# Autodesk Inventor assembly: tower_half
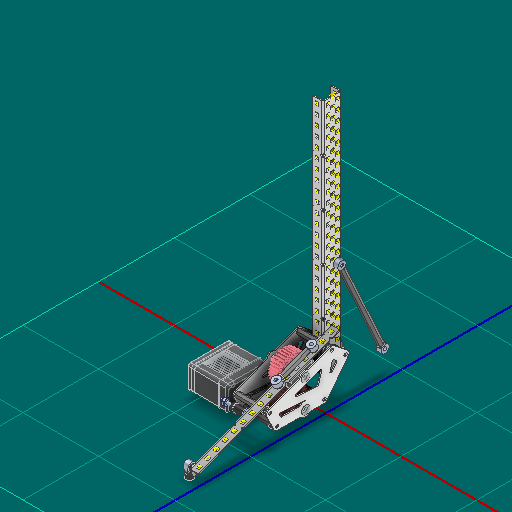
[picture p0: Inventor's stored thumbnail of the model, 512x512]
Saved by Autodesk Inventor 2025 (Build 290162000, 162)
## iProperties
Created: 2024-06-30
Part Number: tower_half
Document SubType Name: Assembly
Designer: Averey Ku
Author: Averey Ku
## Documents named in this file (25)
- C:\Users\avere\vex_robotics_high_stakes\hardware\cad\EARLY_SEASON\tower\tower_half.iam
- C:\Users\avere\vex_robotics_high_stakes\hardware\cad\VEX-CAD-Inventor\Structure\C Channel\Aluminum 1x2x1\Alu C 1x2x1x25.ipt
- C:\Users\avere\vex_robotics_high_stakes\hardware\cad\VEX-CAD-Inventor\Structure\C Channel\Aluminum 2x2x2\Alu C 2x2x2x1.ipt
- C:\Users\avere\vex_robotics_high_stakes\hardware\cad\VEX-CAD-Inventor\Structure\Gussets\C Channel Coupler.ipt
- C:\Users\avere\vex_robotics_high_stakes\hardware\cad\VEX-CAD-Inventor\Motion\Shaft LS\Shaft Collar ipts\Shaft Collar No Screw.ipt
- C:\Users\avere\vex_robotics_high_stakes\hardware\cad\VEX-CAD-Inventor\Motion\Spacers\Washer Steel\SWasher .375 OD x .015625.ipt
- C:\Users\avere\vex_robotics_high_stakes\hardware\cad\VEX-CAD-Inventor\Structure\Standoff\Standoff 5.00.ipt
- C:\Users\avere\vex_robotics_high_stakes\hardware\cad\VEX-CAD-Inventor\Motion\Spacers\Washer Teflon\TWasher .375 OD x .06250.ipt
- C:\Users\avere\vex_robotics_high_stakes\hardware\cad\VEX-CAD-Inventor\Structure\Angle\Aluminum 1x1\Alu Angle 1x1x16.ipt
- C:\Users\avere\vex_robotics_high_stakes\hardware\cad\VEX-CAD-Inventor\Motion\Spacers\Spacer Nylon .375 OD\NSpacer .375 OD x .125.ipt
- C:\Users\avere\vex_robotics_high_stakes\hardware\cad\VEX-CAD-Inventor\Motion\Spacers\Spacer Nylon .375 OD\NSpacer .375 OD x .250.ipt
- C:\Users\avere\vex_robotics_high_stakes\hardware\cad\VEX-CAD-Inventor\Motion\Spacers\Washer Teflon\TWasher .375 OD x .04000.ipt
- C:\Users\avere\vex_robotics_high_stakes\hardware\cad\VEX-CAD-Inventor\Motion\Spacers\Washer Teflon\TWasher .375 OD x .03125.ipt
- C:\Users\avere\vex_robotics_high_stakes\hardware\cad\VEX-CAD-Inventor\Structure\Standoff\Standoff 1.50.ipt
- C:\Users\avere\vex_robotics_high_stakes\hardware\cad\VEX-CAD-Inventor\Motion\Shaft HS\HS Pillow Bearing Block.ipt
- C:\Users\avere\vex_robotics_high_stakes\hardware\cad\EARLY_SEASON\tower\intake_gearbox.iam
- C:\Users\avere\vex_robotics_high_stakes\hardware\cad\VEX-CAD-Inventor\Structure\Hardware\Nut Keps.ipt
- C:\Users\avere\vex_robotics_high_stakes\hardware\cad\VEX-CAD-Inventor\Structure\Hardware\Screw Steel - Star\SScrew Star Smooth 1.500.ipt
- C:\Users\avere\vex_robotics_high_stakes\hardware\cad\VEX-CAD-Inventor\Motion\Spacers\Spacer Nylon .375 OD\NSpacer .375 OD x .500.ipt
- C:\Users\avere\vex_robotics_high_stakes\hardware\cad\VEX-CAD-Inventor\Structure\Hardware\Nut Thin Nylock.ipt
- C:\Users\avere\vex_robotics_high_stakes\hardware\cad\VEX-CAD-Inventor\Motion\Spacers\Washer Steel.ipt
- C:\Users\avere\vex_robotics_high_stakes\hardware\cad\VEX-CAD-Inventor\Structure\Standoff.ipt
- C:\Users\avere\vex_robotics_high_stakes\hardware\cad\VEX-CAD-Inventor\Motion\Spacers\Washer Teflon.ipt
- C:\Users\avere\vex_robotics_high_stakes\hardware\cad\VEX-CAD-Inventor\Motion\Spacers\Spacer Nylon .375 OD.ipt
- C:\Users\avere\vex_robotics_high_stakes\hardware\cad\VEX-CAD-Inventor\Structure\Hardware\Screw Steel - Star.ipt
## Components (30 placed, 19 different names)
1. Alu C 1x2x1x25:1 — Insert:1, Mate:1, Insert:2, Mate:2, Insert:3, Insert:11, Angle:1
2. Alu C 2x2x2x1:1 — Insert:1, Mate:1
3. C Channel Coupler:1 — Insert:2, Mate:2, Insert:36
4. Shaft Collar No Screw:1 — Mate:3, Insert:35
5. SWasher .375 OD x .015625:1 — Insert:5, Insert:35
6. Standoff 5.00:1 — Insert:4, Insert:5
7. Shaft Collar No Screw:2 — Insert:3, Mate:3, Insert:4
8. TWasher .375 OD x .06250:1 — Insert:12
9. Alu Angle 1x1x16:1 — Insert:11, Insert:12, Angle:1, Insert:16, Insert:17, Insert:18, Mate:7, Mate:8, Insert:38, Insert:39, Insert:40
10. Shaft Collar No Screw:3 — Insert:13
11. NSpacer .375 OD x .125:1
12. NSpacer .375 OD x .250:2
13. TWasher .375 OD x .04000:2
14. TWasher .375 OD x .03125:3
15. SWasher .375 OD x .015625:2 — Insert:13
16. Shaft Collar No Screw:4 — Insert:17, Insert:37
17. Shaft Collar No Screw:5 — Insert:16
18. TWasher .375 OD x .06250:4
19. Standoff 1.50:2
20. HS Pillow Bearing Block:1 — Insert:18, Mate:7
21. intake_gearbox:1 [sub-assembly] — Insert:36, Mate:8
22. NSpacer .375 OD x .125:3 — Insert:38
23. NSpacer .375 OD x .125:4 — Insert:37
24. Nut Keps:1 — Insert:39, Insert:44
25. SScrew Star Smooth 1.500:1 — Insert:40
26. NSpacer .375 OD x .500:5 — Insert:43, Insert:44
27. TWasher .375 OD x .04000:5 — Insert:42, Insert:45
28. TWasher .375 OD x .06250:6 — Insert:41, Insert:43
29. TWasher .375 OD x .04000:7 — Insert:41, Insert:42
30. Nut Thin Nylock:1 — Insert:45
## Relationships (38: Insert 29, Mate 8, Angle 1)
- Insert:1: Alu C 1x2x1x25:1 ↔ Alu C 2x2x2x1:1
- Mate:1: Alu C 1x2x1x25:1 ↔ Alu C 2x2x2x1:1
- Insert:2: Alu C 1x2x1x25:1 ↔ C Channel Coupler:1
- Mate:2: Alu C 1x2x1x25:1 ↔ C Channel Coupler:1
- Insert:3: Alu C 1x2x1x25:1 ↔ Shaft Collar No Screw:2
- Mate:3: Shaft Collar No Screw:1 ↔ Shaft Collar No Screw:2
- Insert:4: Standoff 5.00:1 ↔ Shaft Collar No Screw:2
- Insert:5: SWasher .375 OD x .015625:1 ↔ Standoff 5.00:1
- [Mate]: Alu Angle 1x1x16:1 ↔ Shaft Collar No Screw:3
- [Insert]: TWasher .375 OD x .06250:1 ↔ NSpacer .375 OD x .125:1
- [Insert]: Shaft Collar No Screw:3 ↔ NSpacer .375 OD x .125:1
- [Insert]: TWasher .375 OD x .03125:3 ↔ SWasher .375 OD x .015625:2
- [Insert]: TWasher .375 OD x .04000:2 ↔ TWasher .375 OD x .03125:3
- [Insert]: NSpacer .375 OD x .250:2 ↔ TWasher .375 OD x .04000:2
- Insert:11: Alu C 1x2x1x25:1 ↔ Alu Angle 1x1x16:1
- Insert:12: TWasher .375 OD x .06250:1 ↔ Alu Angle 1x1x16:1
- Insert:13: Shaft Collar No Screw:3 ↔ SWasher .375 OD x .015625:2
- Angle:1 (248.9605 deg): Alu C 1x2x1x25:1 ↔ Alu Angle 1x1x16:1
- [Mate]: Shaft Collar No Screw:4 ↔ Shaft Collar No Screw:5
- [Mate]: Shaft Collar No Screw:4 ↔ Shaft Collar No Screw:5
- [Insert]: Shaft Collar No Screw:4 ↔ TWasher .375 OD x .06250:4
- [Insert]: TWasher .375 OD x .06250:4 ↔ Standoff 1.50:2
- Insert:16 (3.175 mm): Alu Angle 1x1x16:1 ↔ Shaft Collar No Screw:5
- Insert:17 (3.175 mm): Alu Angle 1x1x16:1 ↔ Shaft Collar No Screw:4
- Insert:18: Alu Angle 1x1x16:1 ↔ HS Pillow Bearing Block:1
- Mate:7: Alu Angle 1x1x16:1 ↔ HS Pillow Bearing Block:1
- Insert:35 (0.1385 mm): Shaft Collar No Screw:1 ↔ SWasher .375 OD x .015625:1
- Insert:36 (12.7 mm): C Channel Coupler:1 ↔ intake_gearbox:1
- Mate:8: Alu Angle 1x1x16:1 ↔ intake_gearbox:1
- Insert:37: Shaft Collar No Screw:4 ↔ NSpacer .375 OD x .125:4
- Insert:38: Alu Angle 1x1x16:1 ↔ NSpacer .375 OD x .125:3
- Insert:39: Alu Angle 1x1x16:1 ↔ Nut Keps:1
- Insert:40: Alu Angle 1x1x16:1 ↔ SScrew Star Smooth 1.500:1
- Insert:41: TWasher .375 OD x .06250:6 ↔ TWasher .375 OD x .04000:7
- Insert:42: TWasher .375 OD x .04000:5 ↔ TWasher .375 OD x .04000:7
- Insert:43: NSpacer .375 OD x .500:5 ↔ TWasher .375 OD x .06250:6
- Insert:44: Nut Keps:1 ↔ NSpacer .375 OD x .500:5
- Insert:45 (8.4741 mm): TWasher .375 OD x .04000:5 ↔ Nut Thin Nylock:1
